# Autodesk Inventor assembly: sestava tělo estonsko s plechem celý spodek
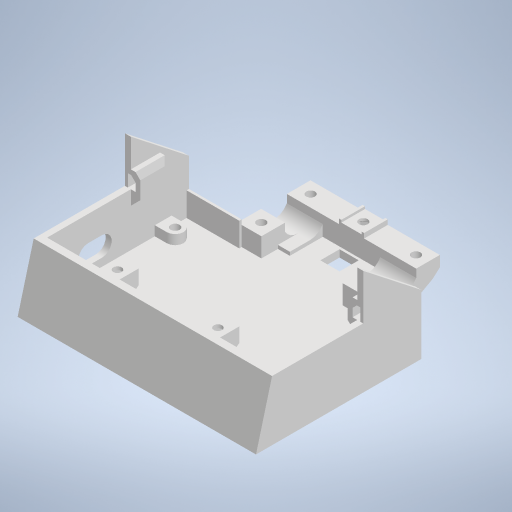
[picture p0: Inventor's stored thumbnail of the model, 512x512]
Saved by Autodesk Inventor 2024 (Build 280153000, 153)
## iProperties
Created: 2023-11-06
Part Number: sestava tělo estonsko s plechem celý spodek
Document SubType Name: Assembly
Designer: jaryj
Author: jaryj
## Documents named in this file (3)
- C:\Users\jaryj\Desktop\Škola\Mini sumo\RoboCop\- 3D -\wip\Tělo s plechem\sestava tělo estonsko s plechem celý spodek.iam
- C:\Users\jaryj\Desktop\Škola\Mini sumo\RoboCop\- 3D -\wip\Tělo s plechem\Plech pro celý spodek.ipt
- C:\Users\jaryj\Desktop\Škola\Mini sumo\RoboCop\- 3D -\wip\Tělo s plechem\tělo estonsko s plechem celý spodek.ipt
## Components (2 placed, 2 different names)
1. Plech pro celý spodek:1 — Tuhé:1
2. tělo estonsko s plechem celý spodek:1 — Tuhé:1
## Relationships (1: WeldJoint 1)
- Tuhé:1 [WeldJoint]: Plech pro celý spodek:1 ↔ tělo estonsko s plechem celý spodek:1
